# Autodesk Inventor assembly: traction_wheel
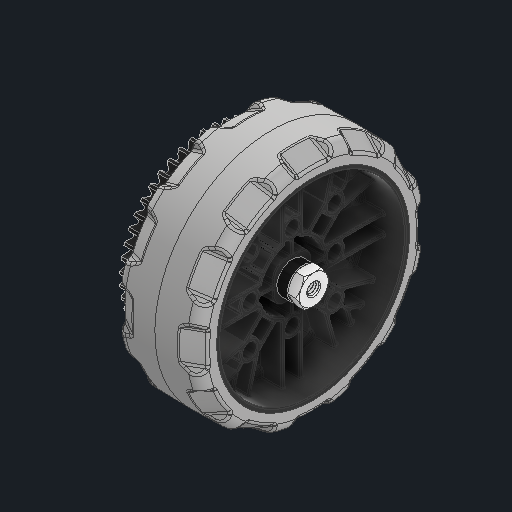
[picture p0: Inventor's stored thumbnail of the model, 512x512]
Saved by Autodesk Inventor 2024 (Build 280153000, 153)
## iProperties
Created: 2023-10-18
Part Number: traction_wheel
Document SubType Name: Assembly
Designer: Averey Ku
Author: Averey Ku
## Documents named in this file (8)
- D:\vex_robotics\hardware\cad\goated_v0.1\chassis\drivebay\traction_wheel.iam
- D:\vex_robotics\hardware\cad\VEX-CAD-Inventor-1.41\Structure\Hardware\Nut Nylon\Nut Nylon - White.ipt
- D:\vex_robotics\hardware\cad\VEX-CAD-Inventor-1.41\Structure\Hardware\Nut Nylon.ipt
- D:\vex_robotics\hardware\cad\VEX-CAD-Inventor-1.41\Motion\Spacers\Spacer Nylon .375 OD\NSpacer .375 OD x .125.ipt
- D:\vex_robotics\hardware\cad\VEX-CAD-Inventor-1.41\Motion\Spacers\Spacer Nylon .375 OD.ipt
- D:\vex_robotics\hardware\cad\VEX-CAD-Inventor-1.41\Motion\Wheels\Traction Wheel\2.75 Traction AS, No Insert.iam
- D:\vex_robotics\hardware\cad\VEX-CAD-Inventor-1.41\Motion\Wheels\Traction Wheel.iam
- D:\vex_robotics\hardware\cad\goated_v0.1\chassis\drivebay\custom_parts\ls_48t.ipt
## Components (4 placed, 4 different names)
1. Nut Nylon - White:1
2. NSpacer .375 OD x .125:1 — Insert:3
3. 2.75 Traction AS, No Insert:1 [sub-assembly] — Insert:2, Insert:3
4. ls_48t:1 — Insert:2
## Relationships (3: Insert 3)
- [Insert]: Nut Nylon - White:1 ↔ NSpacer .375 OD x .125:1
- Insert:2 (3.175 mm): 2.75 Traction AS, No Insert:1 ↔ ls_48t:1
- Insert:3: NSpacer .375 OD x .125:1 ↔ 2.75 Traction AS, No Insert:1
